# Autodesk Inventor assembly: TouchKeyer
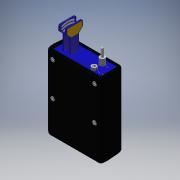
[picture p0: Inventor's stored thumbnail of the model, 180x180]
Saved by Autodesk Inventor 2016 (Build 200138000, 138)
## iProperties
Created: 2016-06-11
Part Number: TouchKeyer
Document SubType Name: Assembly
Designer: Tyler
Author: Tyler
## Documents named in this file (11)
- C:\Users\Tyler\Documents\Small Projects\Personal\morse-practice-oscillator\Mechanicial\Key\TouchKeyer.iam
- C:\Users\Tyler\Documents\Small Projects\Personal\morse-practice-oscillator\Mechanicial\Key\Imported Components\1593P Bottom\1593P Bottom.ipt
- C:\Users\Tyler\Documents\Small Projects\Personal\morse-practice-oscillator\Mechanicial\Key\Imported Components\1593P Battery Cover\1593P Battery Cover.ipt
- C:\Users\Tyler\Documents\Small Projects\Personal\morse-practice-oscillator\Mechanicial\Key\Imported Components\1593P Top\1593P Top.ipt
- C:\Users\Tyler\Documents\Inventor\Content Center Files\R2016\en-US\ANSI B18.6.4(00)\ANSI B18.6.4 - 4-24 - 0.75(41) AB II.ipt
- C:\Users\Tyler\Documents\Small Projects\Personal\morse-practice-oscillator\Mechanicial\Key\AAHolder.ipt
- C:\Users\Tyler\Documents\Small Projects\Personal\morse-practice-oscillator\Mechanicial\Key\AA.ipt
- C:\Users\Tyler\Documents\Small Projects\Personal\morse-practice-oscillator\Mechanicial\Key\KeyerFrontIambic.iam
- C:\Users\Tyler\Documents\Small Projects\Personal\morse-practice-oscillator\Mechanicial\Key\MJ-074N.ipt
- C:\Users\Tyler\Documents\Small Projects\Personal\morse-practice-oscillator\Mechanicial\Key\1MS2.ipt
- C:\Users\Tyler\Documents\Small Projects\Personal\morse-practice-oscillator\Mechanicial\Key\TouchKeyer\AIP\Cable and Harness\TouchKeyer.Harness1.iam
## Components (14 placed, 10 different names)
1. 1593P Bottom:1 — Flush:1, Flush:2, Flush:3, Mate:1, Flush:4, Mate:2, Mate:3, Mate:4, Mate:5, Mate:6, Mate:7, Mate:8, Flush:6, Flush:7, Flush:8, Flush:9, Mate:10, Mate:11, Flush:10
2. 1593P Battery Cover:1 — Mate:1, Flush:4, Flush:5
3. 1593P Top:1 — Mate:2, Mate:3, Mate:4, Mate:9, Mate:12
4. Cross Recessed Flat Countersunk Head Tapping Screw - Type AB - Type II - Inch No. 4 - 24 -  3/4:1 — Mate:6, Flush:6
5. Cross Recessed Flat Countersunk Head Tapping Screw - Type AB - Type II - Inch No. 4 - 24 -  3/4:2 — Mate:5, Flush:8
6. Cross Recessed Flat Countersunk Head Tapping Screw - Type AB - Type II - Inch No. 4 - 24 -  3/4:3 — Mate:7, Flush:7
7. Cross Recessed Flat Countersunk Head Tapping Screw - Type AB - Type II - Inch No. 4 - 24 -  3/4:4 — Mate:8, Flush:9
8. AAHolder:1 — Mate:9, Insert:1, Insert:2, Mate:12
9. AA:1 — Insert:1
10. AA:2 — Insert:2
11. KeyerFrontIambic:1 [sub-assembly] — Mate:10, Mate:11, Flush:10, Insert:3, Angle:1, Insert:5, Angle:2
12. MJ-074N:1 — Insert:3, Angle:1
13. 1MS2:1 — Insert:5, Angle:2
14. Harness1 [sub-assembly]
## Relationships (28: Mate 12, Flush 10, Insert 4, Angle 2)
- Flush:1: 1593P Bottom:1
- Flush:2: 1593P Bottom:1
- Flush:3: 1593P Bottom:1
- Mate:1: 1593P Bottom:1 ↔ 1593P Battery Cover:1
- Flush:4: 1593P Bottom:1 ↔ 1593P Battery Cover:1
- Flush:5: 1593P Battery Cover:1
- Mate:2: 1593P Bottom:1 ↔ 1593P Top:1
- Mate:3: 1593P Bottom:1 ↔ 1593P Top:1
- Mate:4: 1593P Bottom:1 ↔ 1593P Top:1
- Mate:5: 1593P Bottom:1 ↔ Cross Recessed Flat Countersunk Head Tapping Screw - Type AB - Type II - Inch No. 4 - 24 -  3/4:2
- Mate:6: 1593P Bottom:1 ↔ Cross Recessed Flat Countersunk Head Tapping Screw - Type AB - Type II - Inch No. 4 - 24 -  3/4:1
- Mate:7: 1593P Bottom:1 ↔ Cross Recessed Flat Countersunk Head Tapping Screw - Type AB - Type II - Inch No. 4 - 24 -  3/4:3
- Mate:8: 1593P Bottom:1 ↔ Cross Recessed Flat Countersunk Head Tapping Screw - Type AB - Type II - Inch No. 4 - 24 -  3/4:4
- Flush:6: 1593P Bottom:1 ↔ Cross Recessed Flat Countersunk Head Tapping Screw - Type AB - Type II - Inch No. 4 - 24 -  3/4:1
- Flush:7: 1593P Bottom:1 ↔ Cross Recessed Flat Countersunk Head Tapping Screw - Type AB - Type II - Inch No. 4 - 24 -  3/4:3
- Flush:8: 1593P Bottom:1 ↔ Cross Recessed Flat Countersunk Head Tapping Screw - Type AB - Type II - Inch No. 4 - 24 -  3/4:2
- Flush:9: 1593P Bottom:1 ↔ Cross Recessed Flat Countersunk Head Tapping Screw - Type AB - Type II - Inch No. 4 - 24 -  3/4:4
- Mate:9: 1593P Top:1 ↔ AAHolder:1
- Insert:1: AAHolder:1 ↔ AA:1
- Insert:2: AAHolder:1 ↔ AA:2
- Mate:10: 1593P Bottom:1 ↔ KeyerFrontIambic:1
- Mate:11: 1593P Bottom:1 ↔ KeyerFrontIambic:1
- Flush:10: 1593P Bottom:1 ↔ KeyerFrontIambic:1
- Insert:3: KeyerFrontIambic:1 ↔ MJ-074N:1
- Angle:1 (90 deg): KeyerFrontIambic:1 ↔ MJ-074N:1
- Insert:5: KeyerFrontIambic:1 ↔ 1MS2:1
- Angle:2 (0 deg): KeyerFrontIambic:1 ↔ 1MS2:1
- Mate:12: 1593P Top:1 ↔ AAHolder:1
